# Autodesk Inventor assembly: shooter
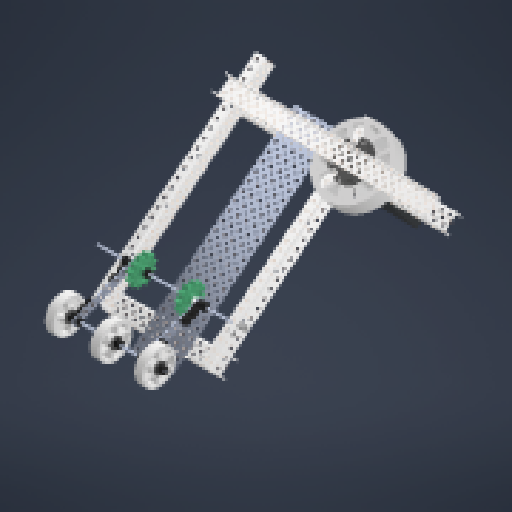
[picture p0: Inventor's stored thumbnail of the model, 512x512]
Saved by Autodesk Inventor 2023 (Build 270158000, 158)
## iProperties
Created: 2023-03-01
Part Number: shooter
Document SubType Name: Assembly
Designer: Windows Macbook
Author: Windows Macbook
## Documents named in this file (18)
- C:\Users\Windows Macbook\Desktop\VRC-SPIN-UP\Inventor\Assembly\Pre Worlds\shooter.iam
- C:\Users\Windows Macbook\Desktop\VRC-SPIN-UP\Inventor\Structure\C Channel\Aluminum 1x2x1\Alu C 1x2x1x14.ipt
- C:\Users\Windows Macbook\Desktop\VRC-SPIN-UP\Inventor\Structure\Plate\Steel\Steel Plate 5x25.ipt
- C:\Users\Windows Macbook\Desktop\VRC-SPIN-UP\Inventor\Motion\Wheels\Flex Wheels\2 Flex, LS.iam
- C:\Users\Windows Macbook\Desktop\VRC-SPIN-UP\Inventor\Motion\Sprockets\9P Sprocket\9P 12T Sprocket, Square.iam
- C:\Users\Windows Macbook\Desktop\VRC-SPIN-UP\Inventor\Motion\Sprockets\9P Sprocket.iam
- C:\Users\Windows Macbook\Desktop\VRC-SPIN-UP\Inventor\Motion\Shaft LS\Shaft LS\Shaft LS 8.0.ipt
- C:\Users\Windows Macbook\Desktop\VRC-SPIN-UP\Inventor\Motion\Shaft LS\Shaft LS.ipt
- C:\Users\Windows Macbook\Desktop\VRC-SPIN-UP\Inventor\Structure\Plate\Steel\Steel Plate 1x8.ipt
- C:\Users\Windows Macbook\Desktop\VRC-SPIN-UP\Inventor\Motion\Shaft LS\Bearing Flat.ipt
- C:\Users\Windows Macbook\Desktop\VRC-SPIN-UP\Inventor\Motion\Spacers\Spacer Nylon .313 OD\NSpacer .313 OD x .250.ipt
- C:\Users\Windows Macbook\Desktop\VRC-SPIN-UP\Inventor\Motion\Spacers\Spacer Nylon .313 OD.ipt
- C:\Users\Windows Macbook\Desktop\VRC-SPIN-UP\Inventor\Motion\Shaft LS\Shaft Collar Rubber.ipt
- C:\Users\Windows Macbook\Desktop\VRC-SPIN-UP\Inventor\Motion\Shaft LS\Shaft LS\Shaft LS 6.5.ipt
- C:\Users\Windows Macbook\Desktop\VRC-SPIN-UP\Inventor\Motion\Wheels\Flex Wheels\4 Flex, LS.iam
- C:\Users\Windows Macbook\Desktop\VRC-SPIN-UP\Inventor\Structure\C Channel\Aluminum 1x2x1\Alu C 1x2x1x25.ipt
- C:\Users\Windows Macbook\Desktop\VRC-SPIN-UP\Inventor\Electronics\V5 Simple Motor.ipt
- C:\Users\Windows Macbook\Desktop\VRC-SPIN-UP\Inventor\Motion\Spacers\Spacer Nylon .313 OD\NSpacer .313 OD x .500.ipt
## Components (37 placed, 14 different names)
1. Alu C 1x2x1x14:1 — Insert:7, Insert:8, Insert:59, Insert:60, Insert:61, Insert:62
2. Alu C 1x2x1x25:1 — Insert:48, Insert:49, Insert:50, Insert:63, Insert:64
3. Steel Plate 5x25:1 — Insert:7, Insert:8
4. 2 Flex, LS:1 [sub-assembly] — Insert:27, Insert:43
5. 9P 12T Sprocket, Square:1 [sub-assembly] — Insert:34, Insert:40
6. 9P 12T Sprocket, Square:3 [sub-assembly] — Insert:23, Insert:38
7. 2 Flex, LS:2 [sub-assembly] — Insert:41, Insert:42, Insert:46
8. Shaft LS 8.0:1
9. Steel Plate 1x8:1 — Insert:21, Insert:22, Insert:24, Insert:25, Insert:26, Insert:47
10. Bearing Flat:1 — Insert:21, Insert:22, Insert:37
11. NSpacer .313 OD x .250:1 — Insert:23, Insert:24
12. Bearing Flat:3 — Insert:25, Insert:26, Insert:27
13. 2 Flex, LS:4 [sub-assembly] — Insert:45
14. Steel Plate 1x8:3 — Insert:41, Insert:44
15. Bearing Flat:4 — Insert:39
16. NSpacer .313 OD x .250:2 — Insert:34
17. Bearing Flat:5
18. Shaft Collar Rubber:1 — Insert:38
19. Shaft Collar Rubber:2 — Insert:37
20. Shaft Collar Rubber:3 — Insert:39
21. Shaft Collar Rubber:4 — Insert:40
22. Shaft Collar Rubber:5 — Insert:42
23. Shaft Collar Rubber:6 — Insert:43, Flush:2, Cylindrical:2
24. Shaft Collar Rubber:7 — Insert:44
25. Shaft Collar Rubber:8 — Insert:47
26. Shaft Collar Rubber:9 — Insert:46
27. Shaft Collar Rubber:10 — Insert:45, Cylindrical:3
28. Shaft LS 6.5:2 — Flush:2, Cylindrical:2, Cylindrical:3
29. 4 Flex, LS:1 [sub-assembly] — Insert:48
30. Bearing Flat:6 — Insert:49, Insert:50, Insert:51, Insert:52, Insert:53
31. Shaft Collar Rubber:11 — Insert:51
32. V5 Simple Motor:1 — Insert:52, Insert:53
33. Alu C 1x2x1x25:2 — Insert:57, Insert:58
34. NSpacer .313 OD x .500:3 — Insert:57, Insert:66
35. NSpacer .313 OD x .500:4 — Insert:58, Insert:65
36. Alu C 1x2x1x25:3 — Insert:61, Insert:62
37. Alu C 1x2x1x25:4 — Insert:59, Insert:60, Insert:63, Insert:64, Insert:65, Insert:66
## Relationships (46: Insert 43, CylindricalJoint 2, Flush 1)
- Insert:7: Alu C 1x2x1x14:1 ↔ Steel Plate 5x25:1
- Insert:8: Alu C 1x2x1x14:1 ↔ Steel Plate 5x25:1
- Insert:21: Steel Plate 1x8:1 ↔ Bearing Flat:1
- Insert:22: Steel Plate 1x8:1 ↔ Bearing Flat:1
- Insert:23: 9P 12T Sprocket, Square:3 ↔ NSpacer .313 OD x .250:1
- Insert:24: Steel Plate 1x8:1 ↔ NSpacer .313 OD x .250:1
- Insert:25: Steel Plate 1x8:1 ↔ Bearing Flat:3
- Insert:26: Steel Plate 1x8:1 ↔ Bearing Flat:3
- Insert:27: 2 Flex, LS:1 ↔ Bearing Flat:3
- [Insert]: Steel Plate 1x8:3 ↔ Bearing Flat:4
- [Insert]: Steel Plate 1x8:3 ↔ Bearing Flat:4
- [Insert]: Steel Plate 1x8:3 ↔ NSpacer .313 OD x .250:2
- [Insert]: Steel Plate 1x8:3 ↔ Bearing Flat:5
- [Insert]: Steel Plate 1x8:3 ↔ Bearing Flat:5
- [Insert]: 2 Flex, LS:4 ↔ Bearing Flat:5
- Insert:34: 9P 12T Sprocket, Square:1 ↔ NSpacer .313 OD x .250:2
- Insert:37 (0.889 mm): Bearing Flat:1 ↔ Shaft Collar Rubber:2
- Insert:38 (0.889 mm): 9P 12T Sprocket, Square:3 ↔ Shaft Collar Rubber:1
- Insert:39 (0.889 mm): Bearing Flat:4 ↔ Shaft Collar Rubber:3
- Insert:40 (0.889 mm): 9P 12T Sprocket, Square:1 ↔ Shaft Collar Rubber:4
- Insert:41 (40.64 mm): 2 Flex, LS:2 ↔ Steel Plate 1x8:3
- Insert:42 (0.889 mm): 2 Flex, LS:2 ↔ Shaft Collar Rubber:5
- Insert:43 (0.889 mm): 2 Flex, LS:1 ↔ Shaft Collar Rubber:6
- Insert:44 (0.889 mm): Steel Plate 1x8:3 ↔ Shaft Collar Rubber:7
- Insert:45 (0.889 mm): 2 Flex, LS:4 ↔ Shaft Collar Rubber:10
- Insert:46 (0.889 mm): 2 Flex, LS:2 ↔ Shaft Collar Rubber:9
- Insert:47 (0.889 mm): Steel Plate 1x8:1 ↔ Shaft Collar Rubber:8
- Flush:2: Shaft Collar Rubber:6 ↔ Shaft LS 6.5:2
- Cylindrical:2: Shaft Collar Rubber:6 ↔ Shaft LS 6.5:2
- Cylindrical:3: Shaft Collar Rubber:10 ↔ Shaft LS 6.5:2
- Insert:48: Alu C 1x2x1x25:1 ↔ 4 Flex, LS:1
- Insert:49: Alu C 1x2x1x25:1 ↔ Bearing Flat:6
- Insert:50: Alu C 1x2x1x25:1 ↔ Bearing Flat:6
- Insert:51 (0.889 mm): Bearing Flat:6 ↔ Shaft Collar Rubber:11
- Insert:52: Bearing Flat:6 ↔ V5 Simple Motor:1
- Insert:53: Bearing Flat:6 ↔ V5 Simple Motor:1
- Insert:57: Alu C 1x2x1x25:2 ↔ NSpacer .313 OD x .500:3
- Insert:58: Alu C 1x2x1x25:2 ↔ NSpacer .313 OD x .500:4
- Insert:59: Alu C 1x2x1x14:1 ↔ Alu C 1x2x1x25:4
- Insert:60: Alu C 1x2x1x14:1 ↔ Alu C 1x2x1x25:4
- Insert:61: Alu C 1x2x1x14:1 ↔ Alu C 1x2x1x25:3
- Insert:62: Alu C 1x2x1x14:1 ↔ Alu C 1x2x1x25:3
- Insert:63: Alu C 1x2x1x25:1 ↔ Alu C 1x2x1x25:4
- Insert:64: Alu C 1x2x1x25:1 ↔ Alu C 1x2x1x25:4
- Insert:65: NSpacer .313 OD x .500:4 ↔ Alu C 1x2x1x25:4
- Insert:66: NSpacer .313 OD x .500:3 ↔ Alu C 1x2x1x25:4
## Named parameters: d33_d26 = 0 mm, d34_d27 = 0 mm, d35_d29 = 0 mm, d36_d30 = 0 mm, d37_d31 = 0 mm, d38_d32 = 0 mm
